# Autodesk Inventor assembly: 529120 DFM-16-150-B-P-A-KF---(0)
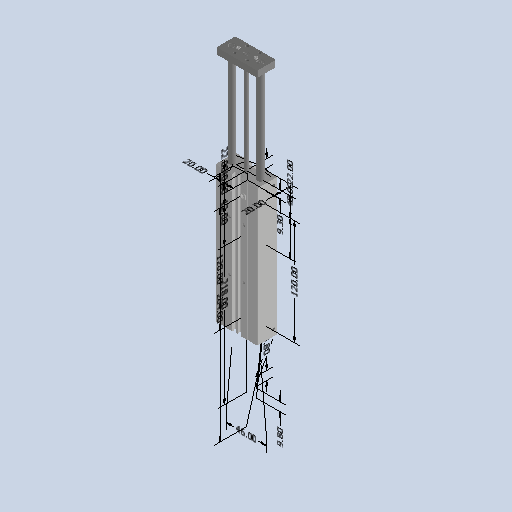
[picture p0: Inventor's stored thumbnail of the model, 512x512]
Saved by Autodesk Inventor 2025.2 (Build 292293000, 293)
## iProperties
Category: PARTsolutions
Company: FESTO
Created: 2025-06-19
Part Number: 529120 DFM-16-150-B-P-A-KF---(0)
Catalog Web Link: www.cadenas.de
Description: DFM-B (m)-Guide cylinder, Modular system
Vendor: FESTO
Document SubType Name: Assembly
Designer: psAdmin
Manufacturer: FESTO
Mass: 1378 g
Surface Area: 1122.99 cm^2
Volume: 425.044 cm^3
Density: 3.24202 g/cm^3
PSOL_IDENT_0: {ATYP=ASSISTANT},{DATA=script=$CADENAS_DATA/23d-libs/festo/webfesto.vbb&M_FAMILY=DFM&M_GROUP=01&M_PA
PSOL_IDENT_1: RTNO=529120&IDCODE1=DFM-16-150-B-P-A-KF&IDCODE2=&C_DFMB_B=B&C_DFMB_DM=16&C_DFMB_HEAD=DFM&M_ABF=A&M_F
PSOL_IDENT_2: HG=KF&N_DFMB_XHUB=150&S_DAR=P&HUB=150&customer_number_cns=&MATES=1&LOD=HI&LOCKERP=0}
NB: 529120 DFM-16-150-B-P-A-KF---(0)
NN: DFM-B (m)
NT: Guide cylinder, Modular system
NBSYN: $TNR. $TYP.$GEWN.-$KDM.-$HUB.-$G.$CUSHT.-A$FT.$S6N.$JT.$ATEXN.$ZUBN.---($HUBST.)
LINA: 529120 DFM-16-150-B-P-A-KF
CATALOG: Festo
TNR: 529120
TYP: DFM
GEW: -
KDM: 16
HUB: 150
HUBST: 0
G: B
CUSH: P
POS: A
F: KF
S6: -
JUST: -
ATEX: -
ZUBS: 0
ZUBG: 0
ZUBI: 0
B1: 67
B2: 65
B3: 45
B4: 4.5
B5: 58
B6: 22
B7: 23
B8: 23.5
B9: 20
B10: 10.5
B11: 46
B12: 9.5
B13: 46
B14: 21.3
B15: 24.4
B16: 33.5
B17: 28
B18: 4
B19: 0
B20: 0
B21: 0
B22: 0
D1: M 5
D2: 7.5
D3: 9
D4: M 5
D5: 5
D6: 4.3
D7: 10
D8: 5
D9: M 4
D10: 6
D11: 0
E1: M5
H1: 32
H2: 30
H3: 26.5
H4: 4
H5: 24
H6: 4
H7: 24
H8: 16
H9: 7.4
H10: 20
H11: 16
H12: 0
H13: 10
H14: 0
L1: 264
L2: 218
L3: 10
L4: 12
L5: 9.8
L6: 9.3
L7: 34
L8: 22
L9: 40
L10: 34
L11: 120
L12: 5
L13: 0
L14: 0
L15: 0
L16: 0
L21: 0
L22: 0
T1: 12
T2: 4.6
T3: 2.1
T4: 10
T5: 1.2
T6: 0
T7: 0
T8: 0
T9: 0
SW2: 10
SW3: 17
SW4: 0
SW5: 0
SW6: 0
SW7: 0
SW8: 0
SW10: 0
CNSMASSEXACT: 1.378
SUPPLIER: FESTO
ARTICLENO: 529120 DFM-16-150-B-P-A-KF---(0)
BOMINFO: 529120 DFM-16-150-B-P-A-KF
CREATOR: CADENAS GmbH
Title: 529120 DFM-16-150-B-P-A-KF
Author: Cadenas PARTsolutions
Comments: Guide cylinder, Modular system
## Documents named in this file (6)
- D:\Useless_Box\CAD-Paspa\Useless Box\Kaufteile\Festo_Fuehrungszylinder150_DFM_16\529120 DFM-16-150-B-P-A-KF---(0).iam
- D:\Useless_Box\CAD-Paspa\Useless Box\Kaufteile\Festo_Fuehrungszylinder150_DFM_16\529120 DFM---16-160-B-P-A-KF---(ZR) 150.ipt
- D:\Useless_Box\CAD-Paspa\Useless Box\Kaufteile\Festo_Fuehrungszylinder150_DFM_16\529120 DFM-16-150-B-P-A-KF---(K).ipt
- D:\Useless_Box\CAD-Paspa\Useless Box\Kaufteile\Festo_Fuehrungszylinder150_DFM_16\8146543 ZBH-5-B.ipt
- D:\Useless_Box\CAD-Paspa\Useless Box\Kaufteile\Festo_Fuehrungszylinder150_DFM_16\8137184 ZBH-9-B.ipt
- D:\Useless_Box\CAD-Paspa\Useless Box\Kaufteile\Festo_Fuehrungszylinder150_DFM_16\DIN-913 - M5x5.ipt
## Components (10 placed, 5 different names)
1. 529120 DFM---16-160-B-P-A-KF---(ZR) 150:1 — zylinder_dfm_XY@1 <-> kolben_dfm_XY@2, zylinder_dfm_Z@1 <-> kolben_dfm_Z@2, zylinder_dfm_YZ@1 <-> kolben_dfm_YZ@2, HUELSE2_1_XY@1 <-> insert_XY@5, HUELSE2_1_Z@1 <-> insert_Z@5, HUELSE2_1_YZ@1 <-> insert_YZ@5, HUELSE2_2_XY@1 <-> insert_XY@6, HUELSE2_2_Z@1 <-> insert_Z@6, HUELSE2_2_YZ@1 <-> insert_YZ@6, HUELSE1_1_XY@1 <-> insert_XY@7, HUELSE1_1_Z@1 <-> insert_Z@7, HUELSE1_1_YZ@1 <-> insert_YZ@7, HUELSE1_2_XY@1 <-> insert_XY@8, HUELSE1_2_Z@1 <-> insert_Z@8, HUELSE1_2_YZ@1 <-> insert_YZ@8, PIN_1_XY@1 <-> IP1_XY@9, PIN_1_Z@1 <-> IP1_Z@9, PIN_1_YZ@1 <-> IP1_YZ@9, PIN_2_XY@1 <-> IP1_XY@10, PIN_2_Z@1 <-> IP1_Z@10, PIN_2_YZ@1 <-> IP1_YZ@10
2. 529120 DFM-16-150-B-P-A-KF---(K):1 — zylinder_dfm_XY@1 <-> kolben_dfm_XY@2, zylinder_dfm_Z@1 <-> kolben_dfm_Z@2, zylinder_dfm_YZ@1 <-> kolben_dfm_YZ@2, HUELSE3_1_XY@2 <-> insert_XY@3, HUELSE3_1_Z@2 <-> insert_Z@3, HUELSE3_1_YZ@2 <-> insert_YZ@3, HUELSE3_2_XY@2 <-> insert_XY@4, HUELSE3_2_Z@2 <-> insert_Z@4, HUELSE3_2_YZ@2 <-> insert_YZ@4
3. 8146543 ZBH-5-B:1 — HUELSE3_1_XY@2 <-> insert_XY@3, HUELSE3_1_Z@2 <-> insert_Z@3, HUELSE3_1_YZ@2 <-> insert_YZ@3
4. 8146543 ZBH-5-B:2 — HUELSE3_2_XY@2 <-> insert_XY@4, HUELSE3_2_Z@2 <-> insert_Z@4, HUELSE3_2_YZ@2 <-> insert_YZ@4
5. 8137184 ZBH-9-B:1 — HUELSE2_1_XY@1 <-> insert_XY@5, HUELSE2_1_Z@1 <-> insert_Z@5, HUELSE2_1_YZ@1 <-> insert_YZ@5
6. 8137184 ZBH-9-B:2 — HUELSE2_2_XY@1 <-> insert_XY@6, HUELSE2_2_Z@1 <-> insert_Z@6, HUELSE2_2_YZ@1 <-> insert_YZ@6
7. 8146543 ZBH-5-B:3 — HUELSE1_1_XY@1 <-> insert_XY@7, HUELSE1_1_Z@1 <-> insert_Z@7, HUELSE1_1_YZ@1 <-> insert_YZ@7
8. 8146543 ZBH-5-B:4 — HUELSE1_2_XY@1 <-> insert_XY@8, HUELSE1_2_Z@1 <-> insert_Z@8, HUELSE1_2_YZ@1 <-> insert_YZ@8
9. DIN-913 - M5x5:1 — PIN_1_XY@1 <-> IP1_XY@9, PIN_1_Z@1 <-> IP1_Z@9, PIN_1_YZ@1 <-> IP1_YZ@9
10. DIN-913 - M5x5:2 — PIN_2_XY@1 <-> IP1_XY@10, PIN_2_Z@1 <-> IP1_Z@10, PIN_2_YZ@1 <-> IP1_YZ@10
## Relationships (27: Mate 16, Angle 9, Flush 2)
- zylinder_dfm_XY@1 <-> kolben_dfm_XY@2 [Mate]: 529120 DFM---16-160-B-P-A-KF---(ZR) 150:1 ↔ 529120 DFM-16-150-B-P-A-KF---(K):1
- zylinder_dfm_Z@1 <-> kolben_dfm_Z@2 [Mate]: 529120 DFM---16-160-B-P-A-KF---(ZR) 150:1 ↔ 529120 DFM-16-150-B-P-A-KF---(K):1
- zylinder_dfm_YZ@1 <-> kolben_dfm_YZ@2 [Angle] (0 deg): 529120 DFM---16-160-B-P-A-KF---(ZR) 150:1 ↔ 529120 DFM-16-150-B-P-A-KF---(K):1
- HUELSE3_1_XY@2 <-> insert_XY@3 [Flush]: 529120 DFM-16-150-B-P-A-KF---(K):1 ↔ 8146543 ZBH-5-B:1
- HUELSE3_1_Z@2 <-> insert_Z@3 [Mate]: 529120 DFM-16-150-B-P-A-KF---(K):1 ↔ 8146543 ZBH-5-B:1
- HUELSE3_1_YZ@2 <-> insert_YZ@3 [Angle] (0 deg): 529120 DFM-16-150-B-P-A-KF---(K):1 ↔ 8146543 ZBH-5-B:1
- HUELSE3_2_XY@2 <-> insert_XY@4 [Flush]: 529120 DFM-16-150-B-P-A-KF---(K):1 ↔ 8146543 ZBH-5-B:2
- HUELSE3_2_Z@2 <-> insert_Z@4 [Mate]: 529120 DFM-16-150-B-P-A-KF---(K):1 ↔ 8146543 ZBH-5-B:2
- HUELSE3_2_YZ@2 <-> insert_YZ@4 [Angle] (0 deg): 529120 DFM-16-150-B-P-A-KF---(K):1 ↔ 8146543 ZBH-5-B:2
- HUELSE2_1_XY@1 <-> insert_XY@5 [Mate]: 529120 DFM---16-160-B-P-A-KF---(ZR) 150:1 ↔ 8137184 ZBH-9-B:1
- HUELSE2_1_Z@1 <-> insert_Z@5 [Mate]: 529120 DFM---16-160-B-P-A-KF---(ZR) 150:1 ↔ 8137184 ZBH-9-B:1
- HUELSE2_1_YZ@1 <-> insert_YZ@5 [Angle] (0 deg): 529120 DFM---16-160-B-P-A-KF---(ZR) 150:1 ↔ 8137184 ZBH-9-B:1
- HUELSE2_2_XY@1 <-> insert_XY@6 [Mate]: 529120 DFM---16-160-B-P-A-KF---(ZR) 150:1 ↔ 8137184 ZBH-9-B:2
- HUELSE2_2_Z@1 <-> insert_Z@6 [Mate]: 529120 DFM---16-160-B-P-A-KF---(ZR) 150:1 ↔ 8137184 ZBH-9-B:2
- HUELSE2_2_YZ@1 <-> insert_YZ@6 [Angle] (0 deg): 529120 DFM---16-160-B-P-A-KF---(ZR) 150:1 ↔ 8137184 ZBH-9-B:2
- HUELSE1_1_XY@1 <-> insert_XY@7 [Mate]: 529120 DFM---16-160-B-P-A-KF---(ZR) 150:1 ↔ 8146543 ZBH-5-B:3
- HUELSE1_1_Z@1 <-> insert_Z@7 [Mate]: 529120 DFM---16-160-B-P-A-KF---(ZR) 150:1 ↔ 8146543 ZBH-5-B:3
- HUELSE1_1_YZ@1 <-> insert_YZ@7 [Angle] (0 deg): 529120 DFM---16-160-B-P-A-KF---(ZR) 150:1 ↔ 8146543 ZBH-5-B:3
- HUELSE1_2_XY@1 <-> insert_XY@8 [Mate]: 529120 DFM---16-160-B-P-A-KF---(ZR) 150:1 ↔ 8146543 ZBH-5-B:4
- HUELSE1_2_Z@1 <-> insert_Z@8 [Mate]: 529120 DFM---16-160-B-P-A-KF---(ZR) 150:1 ↔ 8146543 ZBH-5-B:4
- HUELSE1_2_YZ@1 <-> insert_YZ@8 [Angle] (0 deg): 529120 DFM---16-160-B-P-A-KF---(ZR) 150:1 ↔ 8146543 ZBH-5-B:4
- PIN_1_XY@1 <-> IP1_XY@9 [Mate]: 529120 DFM---16-160-B-P-A-KF---(ZR) 150:1 ↔ DIN-913 - M5x5:1
- PIN_1_Z@1 <-> IP1_Z@9 [Mate]: 529120 DFM---16-160-B-P-A-KF---(ZR) 150:1 ↔ DIN-913 - M5x5:1
- PIN_1_YZ@1 <-> IP1_YZ@9 [Angle] (0 deg): 529120 DFM---16-160-B-P-A-KF---(ZR) 150:1 ↔ DIN-913 - M5x5:1
- PIN_2_XY@1 <-> IP1_XY@10 [Mate]: 529120 DFM---16-160-B-P-A-KF---(ZR) 150:1 ↔ DIN-913 - M5x5:2
- PIN_2_Z@1 <-> IP1_Z@10 [Mate]: 529120 DFM---16-160-B-P-A-KF---(ZR) 150:1 ↔ DIN-913 - M5x5:2
- PIN_2_YZ@1 <-> IP1_YZ@10 [Angle] (0 deg): 529120 DFM---16-160-B-P-A-KF---(ZR) 150:1 ↔ DIN-913 - M5x5:2
